# Autodesk Inventor assembly: ロッド
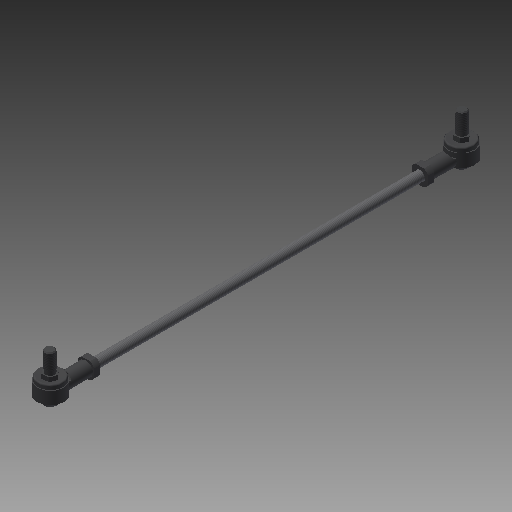
[picture p0: Inventor's stored thumbnail of the model, 512x512]
Saved by Autodesk Inventor 2018 (Build 220112000, 112)
## iProperties
Created: 2017-10-07
Part Number: ロッド
Material: 一般
Document SubType Name: Assembly
Designer: Kosei
Author: Kosei
## Documents named in this file (3)
- D:\Works\RBBR\CAD\ステアリング\ロッド.iam
- D:\Works\RBBR\CAD\ステアリング\ロッド.ipt
- D:\Works\RBBR\CAD\汎用部品\エルボール10mm\LHSA 10.iam
## Components (3 placed, 2 different names)
1. ロッド:1 — リジッド:1, リジッド:2
2. LHSA 10:1 [sub-assembly] — リジッド:1
3. LHSA 10:2 [sub-assembly] — リジッド:2
## Relationships (2: WeldJoint 2)
- リジッド:1 [WeldJoint] (-20 mm): ロッド:1 ↔ LHSA 10:1
- リジッド:2 [WeldJoint] (-20 mm): ロッド:1 ↔ LHSA 10:2
